# Autodesk Inventor assembly: F4C9-204 Top Bearing block
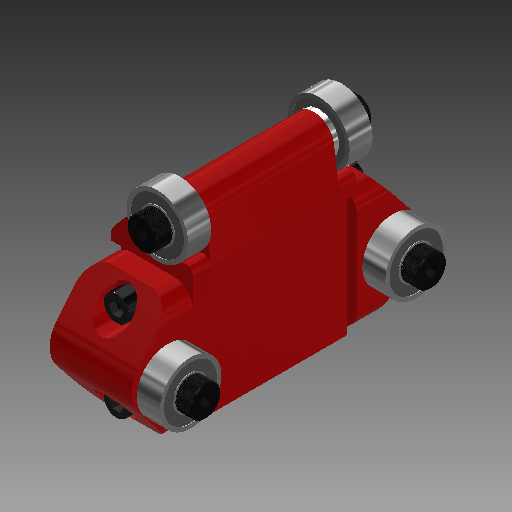
[picture p0: Inventor's stored thumbnail of the model, 512x512]
Saved by Autodesk Inventor 2022 (Build 260153000, 153)
## iProperties
Created: 2020-08-10
Part Number: F4C9-204 Top Bearing block
Document SubType Name: Assembly
## Documents named in this file (12)
- D:\FRC 1369 Minotaur\2020.5 Minotaur\Collaborative Parts Lib\Elevators\Billet Blocks\254 Top Side Bearing Block.iam
- D:\FRC 1369 Minotaur\2020.5 Minotaur\Collaborative Parts Lib\Power Transfer\Bearings\R4A.ipt
- E:\Middleton Robotics\Parts Library\Shaft Accessories\Bearings.ipt
- E:\Middleton Robotics\Parts Library\Hardware\Shoulder Bolt.ipt
- D:\FRC 1369 Minotaur\2020.5 Minotaur\Collaborative Parts Lib\Hardware\Spacers & Standoffs\Aluminum Unthreaded Spacer (0.25in x 0.063Lg x 0.5OD).ipt
- E:\Middleton Robotics\Parts Library\Hardware\Spacers & Standoffs.ipt
- D:\FRC 1369 Minotaur\2020.5 Minotaur\Collaborative Parts Lib\Hardware\Shoulder Bolt\0.25Dia x 0.75 Shoulder Bolt.ipt
- D:\FRC 1369 Minotaur\2020.5 Minotaur\Collaborative Parts Lib\Hardware\Machine Screws\10-32 UNFx0.5 Socket Head Cap Screw.ipt
- E:\Middleton Robotics\Parts Library\Hardware\Machine Screws.ipt
- D:\FRC 1369 Minotaur\2020.5 Minotaur\Collaborative Parts Lib\Hardware\Shoulder Bolt\0.25Dia x 0.5 Shoulder Bolt.ipt
- D:\FRC 1369 Minotaur\2020.5 Minotaur\Collaborative Parts Lib\Elevators\Billet Blocks\254 Top Bearing Block.ipt
- D:\FRC 1369 Minotaur\2020.5 Minotaur\Collaborative Parts Lib\Elevators\Billet Blocks\254 Side Bearing Block.ipt
## Components (19 placed, 7 different names)
1. 254 Top Bearing Block:1 — Insert:10, Insert:11, Insert:12, Insert:13, Insert:20, Insert:22
2. 254 Side Bearing Block:1 — Insert:10, Insert:11, Insert:14, Insert:17
3. R4A:3
4. 0.25Dia x 0.75 Shoulder Bolt:2
5. 254 Side Bearing Block:2 — Insert:12, Insert:13, Insert:15, Insert:16
6. R4A:4
7. 0.25Dia x 0.75 Shoulder Bolt:3
8. Aluminum Unthreaded Spacer (0.25in x 0.063Lg x 0.5OD):1
9. Aluminum Unthreaded Spacer (0.25in x 0.063Lg x 0.5OD):2
10. 10-32 UNFx0.5 Socket Head Cap Screw:1 — Insert:14
11. 10-32 UNFx0.5 Socket Head Cap Screw:2 — Insert:15
12. 10-32 UNFx0.5 Socket Head Cap Screw:3 — Insert:16
13. 10-32 UNFx0.5 Socket Head Cap Screw:4 — Insert:17
14. R4A:5 — Insert:21
15. 0.25Dia x 0.5 Shoulder Bolt:6
16. Aluminum Unthreaded Spacer (0.25in x 0.063Lg x 0.5OD):3 — Insert:20, Insert:21
17. R4A:6 — Insert:23
18. 0.25Dia x 0.5 Shoulder Bolt:7
19. Aluminum Unthreaded Spacer (0.25in x 0.063Lg x 0.5OD):4 — Insert:22, Insert:23
## Relationships (20: Insert 20)
- [Insert]: R4A:3 ↔ 0.25Dia x 0.75 Shoulder Bolt:2
- [Insert] (1.5875 mm): 254 Side Bearing Block:1 ↔ R4A:3
- [Insert]: R4A:4 ↔ 0.25Dia x 0.75 Shoulder Bolt:3
- [Insert] (1.5875 mm): 254 Side Bearing Block:2 ↔ R4A:4
- [Insert]: 254 Side Bearing Block:2 ↔ Aluminum Unthreaded Spacer (0.25in x 0.063Lg x 0.5OD):1
- [Insert]: 254 Side Bearing Block:1 ↔ Aluminum Unthreaded Spacer (0.25in x 0.063Lg x 0.5OD):2
- Insert:10 (1.5875 mm): 254 Top Bearing Block:1 ↔ 254 Side Bearing Block:1
- Insert:11 (1.5875 mm): 254 Top Bearing Block:1 ↔ 254 Side Bearing Block:1
- Insert:12 (1.5875 mm): 254 Top Bearing Block:1 ↔ 254 Side Bearing Block:2
- Insert:13 (1.5875 mm): 254 Top Bearing Block:1 ↔ 254 Side Bearing Block:2
- Insert:14: 254 Side Bearing Block:1 ↔ 10-32 UNFx0.5 Socket Head Cap Screw:1
- Insert:15: 254 Side Bearing Block:2 ↔ 10-32 UNFx0.5 Socket Head Cap Screw:2
- Insert:16: 254 Side Bearing Block:2 ↔ 10-32 UNFx0.5 Socket Head Cap Screw:3
- Insert:17: 254 Side Bearing Block:1 ↔ 10-32 UNFx0.5 Socket Head Cap Screw:4
- [Insert]: R4A:5 ↔ 0.25Dia x 0.5 Shoulder Bolt:6
- [Insert]: R4A:6 ↔ 0.25Dia x 0.5 Shoulder Bolt:7
- Insert:20: 254 Top Bearing Block:1 ↔ Aluminum Unthreaded Spacer (0.25in x 0.063Lg x 0.5OD):3
- Insert:21: R4A:5 ↔ Aluminum Unthreaded Spacer (0.25in x 0.063Lg x 0.5OD):3
- Insert:22: 254 Top Bearing Block:1 ↔ Aluminum Unthreaded Spacer (0.25in x 0.063Lg x 0.5OD):4
- Insert:23: R4A:6 ↔ Aluminum Unthreaded Spacer (0.25in x 0.063Lg x 0.5OD):4
## Named parameters: d95_d71 = 0 mm, d96_d72 = 1.5875 mm, d79_d71 = 0 mm, d80_d72 = 1.5875 mm, d17_d79_d71 = 0 mm, d18_d79_d71 = 0 mm
